# Autodesk Inventor assembly: Overall_Assembly_Rev3
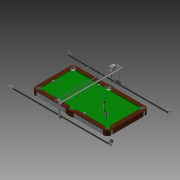
[picture p0: Inventor's stored thumbnail of the model, 180x180]
Saved by Autodesk Inventor 2015 (Build 190159000, 159)
## iProperties
Created: 2017-01-22
Part Number: Overall_Assembly_Rev3
Document SubType Name: Assembly
Designer: Guy
Author: Guy
## Documents named in this file (13)
- C:\Users\1esh9\Documents\Capstone-Project\doc\CAD\LowLevel_Rev3\Overall_Assembly_Rev3.iam
- C:\Users\1esh9\Documents\Capstone-Project\doc\CAD\Pool Table\Table_Model.ipt
- C:\Users\1esh9\Documents\Capstone-Project\doc\CAD\LowLevel_Rev3\X_rail_Assembly_Rev3.iam
- C:\Users\1esh9\Documents\Capstone-Project\doc\CAD\LowLevel_Rev3\Y_rail_Assembly_Rev3.iam
- C:\Users\1esh9\Documents\Capstone-Project\doc\CAD\LowLevel_Rev2\Pool_Ball_Stripe.ipt
- C:\Users\1esh9\Documents\Capstone-Project\doc\CAD\Nuts and Bolts\1-2in_13tpi x 8 in.ipt
- C:\Users\1esh9\Documents\Capstone-Project\doc\CAD\SM2\Overall_Shooting_Mechanism2.iam
- C:\Users\1esh9\Documents\Capstone-Project\doc\CAD\Stepper Motor\NEMA-17\NEMA 17 with T5 Pulley.iam
- C:\Users\1esh9\Documents\Capstone-Project\doc\CAD\Stepper Motor\NEMA-17\holder.ipt
- C:\Users\1esh9\Documents\Capstone-Project\doc\CAD\LowLevel_Rev3\Arm_Pulley_Connector.ipt
- C:\Users\1esh9\Documents\Capstone-Project\doc\CAD\LowLevel_Rev3\XY_Wheel-SquareBar-Rev3.ipt
- C:\Users\1esh9\Documents\Capstone-Project\doc\CAD\LowLevel_Rev3\Arm-Belt-Holder.ipt
- C:\Users\1esh9\Documents\Capstone-Project\doc\CAD\Stepper Motor\NEMA 23\NEMA 23.ipt
## Components (19 placed, 12 different names)
1. Table_Model:1 — Tangent:1, Tangent:2, Tangent:3, Tangent:4, Tangent:5, Tangent:6, Mate:49, Mate:52, Mate:57, Mate:58, Mate:80, Mate:83, Tangent:7, Angle:1
2. Pool_Ball_Stripe:1 — Tangent:1, Tangent:2
3. Pool_Ball_Stripe:2 — Tangent:3, Tangent:4
4. Pool_Ball_Stripe:3 — Tangent:5, Tangent:6
5. 1-2in_13tpi x 8 in:1 — Mate:57, Mate:71, Mate:81
6. 1-2in_13tpi x 8 in:2 — Mate:58, Mate:69, Mate:70
7. 1-2in_13tpi x 8 in:3 — Mate:49, Mate:76, Mate:77
8. 1-2in_13tpi x 8 in:4 — Mate:52, Mate:74, Mate:75
9. holder:1 — Mate:97, Mate:98, Mate:99, Mate:100, Mate:101, Angle:2, Mate:102, Mate:103
10. X_rail_Assembly_Rev3:1 [sub-assembly] — Mate:69, Mate:70, Mate:71, Mate:80, Mate:81, Flush:1, Mate:85, Mate:91, Mate:92, Mate:93, Mate:94, Mate:104, Mate:105, Mate:106, Mate:109, Mate:110, Mate:111, Mate:115, Mate:116, Mate:117, Mate:118, Angle:3
11. X_rail_Assembly_Rev3:2 [sub-assembly] — Mate:74, Mate:75, Mate:76, Mate:77, Mate:83, Angle:1, Flush:1, Mate:86, Mate:99, Mate:100, Mate:101, Mate:102, Mate:103, Mate:112, Mate:113, Mate:114
12. Overall_Shooting_Mechanism2:1 [sub-assembly] — Tangent:7
13. Y_rail_Assembly_Rev3:1 [sub-assembly] — Mate:85, Mate:86, Mate:91, Mate:92, Mate:93, Mate:94
14. NEMA 17 with T5 Pulley:1 [sub-assembly] — Mate:97, Mate:98, Angle:2
15. Arm_Pulley_Connector:1 — Mate:104, Mate:105, Mate:106, Mate:107, Mate:108, Mate:118, Angle:3
16. XY_Wheel-SquareBar-Rev3:1 — Mate:107, Mate:108
17. Arm-Belt-Holder:1 — Mate:109, Mate:110, Mate:111
18. Arm-Belt-Holder:2 — Mate:112, Mate:113, Mate:114
19. NEMA 23:1 — Mate:115, Mate:116, Mate:117
## Relationships (53: Mate 42, Tangent 7, Angle 3, Flush 1)
- Tangent:1: Table_Model:1 ↔ Pool_Ball_Stripe:1
- Tangent:2: Table_Model:1 ↔ Pool_Ball_Stripe:1
- Tangent:3: Table_Model:1 ↔ Pool_Ball_Stripe:2
- Tangent:4: Table_Model:1 ↔ Pool_Ball_Stripe:2
- Tangent:5: Table_Model:1 ↔ Pool_Ball_Stripe:3
- Tangent:6: Table_Model:1 ↔ Pool_Ball_Stripe:3
- Mate:49: Table_Model:1 ↔ 1-2in_13tpi x 8 in:3
- Mate:52: Table_Model:1 ↔ 1-2in_13tpi x 8 in:4
- Mate:57: Table_Model:1 ↔ 1-2in_13tpi x 8 in:1
- Mate:58: Table_Model:1 ↔ 1-2in_13tpi x 8 in:2
- Mate:69: 1-2in_13tpi x 8 in:2 ↔ X_rail_Assembly_Rev3:1
- Mate:70: 1-2in_13tpi x 8 in:2 ↔ X_rail_Assembly_Rev3:1
- Mate:71: 1-2in_13tpi x 8 in:1 ↔ X_rail_Assembly_Rev3:1
- Mate:74: 1-2in_13tpi x 8 in:4 ↔ X_rail_Assembly_Rev3:2
- Mate:75: 1-2in_13tpi x 8 in:4 ↔ X_rail_Assembly_Rev3:2
- Mate:76: 1-2in_13tpi x 8 in:3 ↔ X_rail_Assembly_Rev3:2
- Mate:77: 1-2in_13tpi x 8 in:3 ↔ X_rail_Assembly_Rev3:2
- Mate:80 (220 mm): Table_Model:1 ↔ X_rail_Assembly_Rev3:1
- Mate:81: 1-2in_13tpi x 8 in:1 ↔ X_rail_Assembly_Rev3:1
- Mate:83 (201 mm): Table_Model:1 ↔ X_rail_Assembly_Rev3:2
- Tangent:7: Table_Model:1 ↔ Overall_Shooting_Mechanism2:1
- Angle:1 (0 deg): Table_Model:1 ↔ X_rail_Assembly_Rev3:2
- Flush:1: X_rail_Assembly_Rev3:1 ↔ X_rail_Assembly_Rev3:2
- Mate:85: X_rail_Assembly_Rev3:1 ↔ Y_rail_Assembly_Rev3:1
- Mate:86: X_rail_Assembly_Rev3:2 ↔ Y_rail_Assembly_Rev3:1
- Mate:91: X_rail_Assembly_Rev3:1 ↔ Y_rail_Assembly_Rev3:1
- Mate:92: X_rail_Assembly_Rev3:1 ↔ Y_rail_Assembly_Rev3:1
- Mate:93: X_rail_Assembly_Rev3:1 ↔ Y_rail_Assembly_Rev3:1
- Mate:94: X_rail_Assembly_Rev3:1 ↔ Y_rail_Assembly_Rev3:1
- Mate:97: holder:1 ↔ NEMA 17 with T5 Pulley:1
- Mate:98: holder:1 ↔ NEMA 17 with T5 Pulley:1
- Mate:99: holder:1 ↔ X_rail_Assembly_Rev3:2
- Mate:100: holder:1 ↔ X_rail_Assembly_Rev3:2
- Mate:101: holder:1 ↔ X_rail_Assembly_Rev3:2
- Angle:2 (0 deg): holder:1 ↔ NEMA 17 with T5 Pulley:1
- Mate:102: holder:1 ↔ X_rail_Assembly_Rev3:2
- Mate:103: holder:1 ↔ X_rail_Assembly_Rev3:2
- Mate:104: X_rail_Assembly_Rev3:1 ↔ Arm_Pulley_Connector:1
- Mate:105: X_rail_Assembly_Rev3:1 ↔ Arm_Pulley_Connector:1
- Mate:106: X_rail_Assembly_Rev3:1 ↔ Arm_Pulley_Connector:1
- Mate:107: Arm_Pulley_Connector:1 ↔ XY_Wheel-SquareBar-Rev3:1
- Mate:108 (3.75 mm): Arm_Pulley_Connector:1 ↔ XY_Wheel-SquareBar-Rev3:1
- Mate:109: X_rail_Assembly_Rev3:1 ↔ Arm-Belt-Holder:1
- Mate:110: X_rail_Assembly_Rev3:1 ↔ Arm-Belt-Holder:1
- Mate:111: X_rail_Assembly_Rev3:1 ↔ Arm-Belt-Holder:1
- Mate:112: X_rail_Assembly_Rev3:2 ↔ Arm-Belt-Holder:2
- Mate:113: X_rail_Assembly_Rev3:2 ↔ Arm-Belt-Holder:2
- Mate:114: X_rail_Assembly_Rev3:2 ↔ Arm-Belt-Holder:2
- Mate:115: X_rail_Assembly_Rev3:1 ↔ NEMA 23:1
- Mate:116: X_rail_Assembly_Rev3:1 ↔ NEMA 23:1
- Mate:117: X_rail_Assembly_Rev3:1 ↔ NEMA 23:1
- Mate:118: X_rail_Assembly_Rev3:1 ↔ Arm_Pulley_Connector:1
- Angle:3 (0 deg): X_rail_Assembly_Rev3:1 ↔ Arm_Pulley_Connector:1
